# Autodesk Inventor assembly: Gameboard
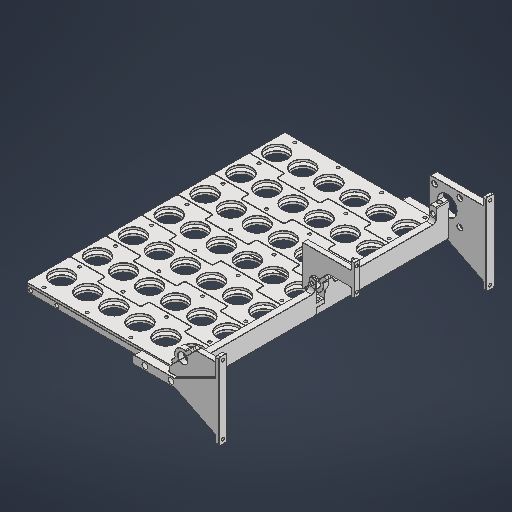
[picture p0: Inventor's stored thumbnail of the model, 512x512]
Saved by Autodesk Inventor 2025 (Build 290162010, 162A)
## iProperties
Created: 2025-12-04
Part Number: Gameboard
Document SubType Name: Assembly
Designer: FizzyApple12
Author: FizzyApple12
## Documents named in this file (10)
- C:\Users\FizzyApple12\Desktop\connect-4-robot\mcad\Gameboard\Gameboard.iam
- C:\Users\FizzyApple12\Desktop\connect-4-robot\mcad\Gameboard\Chute-Half.ipt
- C:\Users\FizzyApple12\Desktop\connect-4-robot\mcad\Gameboard\Backer.ipt
- C:\Users\FizzyApple12\Desktop\connect-4-robot\mcad\Gameboard\Backer-End.ipt
- C:\Users\FizzyApple12\Desktop\connect-4-robot\mcad\Gameboard\Board-Stand-Motor.ipt
- C:\Users\FizzyApple12\Desktop\connect-4-robot\mcad\Gameboard\Half-Shaft-Motor.ipt
- C:\Users\FizzyApple12\Desktop\connect-4-robot\mcad\Gameboard\Board-Stand-Idler.ipt
- C:\Users\FizzyApple12\Desktop\connect-4-robot\mcad\Gameboard\Idler-Clamp.ipt
- C:\Users\FizzyApple12\Desktop\connect-4-robot\mcad\Gameboard\Half-Shaft-Idler.ipt
- C:\Users\FizzyApple12\Desktop\connect-4-robot\mcad\Gameboard\Board-Stand-Center.ipt
## Components (16 placed, 9 different names)
1. Chute-Half:1 — Flush:1, Flush:2, Mate:7, Mate:10, Mate:11, Mate:15, Mate:16, Mate:17, Mate:18, Mate:26, Mate:27, Mate:28, Mate:29, Mate:30, Mate:31
2. Chute-Half:2 — Flush:1, Flush:2, Mate:5, Mate:6, Mate:8, Mate:9, Mate:19, Mate:20, Mate:21, Mate:22, Mate:23, Mate:24, Mate:25, Mate:34, Mate:35, Mate:36
3. Backer:2 — Mate:5, Mate:6, Mate:7
4. Backer:3 — Mate:8, Mate:21, Mate:22
5. Backer:4 — Mate:9, Mate:19, Mate:20
6. Backer:5 — Mate:10, Mate:17, Mate:18
7. Backer:6 — Mate:11, Mate:15, Mate:16
8. Backer-End:1 — Mate:26, Mate:27, Mate:28
9. Backer-End:2 — Mate:23, Mate:24, Mate:25
10. Board-Stand-Motor:1 — Mate:29, Mate:30, Mate:31, Mate:32, Mate:33
11. Half-Shaft-Motor:1 — Mate:32, Mate:33, Mate:41, Mate:42, Mate:43
12. Board-Stand-Idler:1 — Mate:34, Mate:35, Mate:36, Mate:37, Mate:38, Mate:39, Mate:40, Flush:3
13. Idler-Clamp:1 — Mate:37, Mate:38, Mate:39
14. Half-Shaft-Idler:1 — Mate:40, Mate:41
15. Idler-Clamp:2 — Mate:42, Mate:44
16. Board-Stand-Center:1 — Mate:43, Mate:44, Flush:3
## Relationships (40: Mate 37, Flush 3)
- Flush:1: Chute-Half:1 ↔ Chute-Half:2
- Flush:2: Chute-Half:1 ↔ Chute-Half:2
- Mate:5: Chute-Half:2 ↔ Backer:2
- Mate:6: Chute-Half:2 ↔ Backer:2
- Mate:7: Chute-Half:1 ↔ Backer:2
- Mate:8: Chute-Half:2 ↔ Backer:3
- Mate:9: Chute-Half:2 ↔ Backer:4
- Mate:10: Chute-Half:1 ↔ Backer:5
- Mate:11: Chute-Half:1 ↔ Backer:6
- Mate:15: Chute-Half:1 ↔ Backer:6
- Mate:16: Chute-Half:1 ↔ Backer:6
- Mate:17: Chute-Half:1 ↔ Backer:5
- Mate:18: Chute-Half:1 ↔ Backer:5
- Mate:19: Chute-Half:2 ↔ Backer:4
- Mate:20: Chute-Half:2 ↔ Backer:4
- Mate:21: Chute-Half:2 ↔ Backer:3
- Mate:22: Chute-Half:2 ↔ Backer:3
- Mate:23: Chute-Half:2 ↔ Backer-End:2
- Mate:24: Chute-Half:2 ↔ Backer-End:2
- Mate:25: Chute-Half:2 ↔ Backer-End:2
- Mate:26: Chute-Half:1 ↔ Backer-End:1
- Mate:27: Chute-Half:1 ↔ Backer-End:1
- Mate:28: Chute-Half:1 ↔ Backer-End:1
- Mate:29: Chute-Half:1 ↔ Board-Stand-Motor:1
- Mate:30: Chute-Half:1 ↔ Board-Stand-Motor:1
- Mate:31: Chute-Half:1 ↔ Board-Stand-Motor:1
- Mate:32 (-25.4 mm): Board-Stand-Motor:1 ↔ Half-Shaft-Motor:1
- Mate:33: Board-Stand-Motor:1 ↔ Half-Shaft-Motor:1
- Mate:34: Chute-Half:2 ↔ Board-Stand-Idler:1
- Mate:35: Chute-Half:2 ↔ Board-Stand-Idler:1
- Mate:36: Chute-Half:2 ↔ Board-Stand-Idler:1
- Mate:37: Board-Stand-Idler:1 ↔ Idler-Clamp:1
- Mate:38: Board-Stand-Idler:1 ↔ Idler-Clamp:1
- Mate:39: Board-Stand-Idler:1 ↔ Idler-Clamp:1
- Mate:40: Board-Stand-Idler:1 ↔ Half-Shaft-Idler:1
- Mate:41: Half-Shaft-Motor:1 ↔ Half-Shaft-Idler:1
- Mate:42: Half-Shaft-Motor:1 ↔ Idler-Clamp:2
- Mate:43: Half-Shaft-Motor:1 ↔ Board-Stand-Center:1
- Mate:44: Idler-Clamp:2 ↔ Board-Stand-Center:1
- Flush:3: Board-Stand-Idler:1 ↔ Board-Stand-Center:1
